# Autodesk Inventor assembly: Case
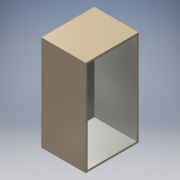
[picture p0: Inventor's stored thumbnail of the model, 180x180]
Saved by Autodesk Inventor 2017 (Build 210142000, 142)
## iProperties
Created: 2016-12-13
Part Number: Case
Document SubType Name: Assembly
Designer: umr
Author: umr
## Documents named in this file (4)
- D:\SeniorProject\Models2\Case\Case.iam
- D:\SeniorProject\Models2\Case\NarrowWall.iam
- D:\SeniorProject\Models2\Case\WideWall.iam
- D:\SeniorProject\Models2\Case\Ceiling.iam
## Components (5 placed, 3 different names)
1. NarrowWall:1 [sub-assembly] — Mate:2, Flush:7, Flush:14, Flush:16, Mate:6, Flush:17, Animation1
2. NarrowWall:2 [sub-assembly] — Flush:12, Flush:13, Animation2
3. WideWall:1 [sub-assembly] — Mate:2, Flush:7, Flush:12, Flush:13, Flush:14, Flush:18, Animation3
4. WideWall:2 [sub-assembly] — Flush:16, Mate:6, Animation1, Animation2
5. Ceiling:1 [sub-assembly] — Flush:17, Flush:18, Animation3
## Relationships (12: Flush 8, Mate 4)
- Mate:2: NarrowWall:1 ↔ WideWall:1
- Flush:7: NarrowWall:1 ↔ WideWall:1
- Flush:12: NarrowWall:2 ↔ WideWall:1
- Flush:13: NarrowWall:2 ↔ WideWall:1
- Flush:14: NarrowWall:1 ↔ WideWall:1
- Flush:16: NarrowWall:1 ↔ WideWall:2
- Mate:6: NarrowWall:1 ↔ WideWall:2
- Flush:17: NarrowWall:1 ↔ Ceiling:1
- Flush:18: WideWall:1 ↔ Ceiling:1
- Animation1 [Flush]: NarrowWall:1 ↔ WideWall:2
- Animation2 [Mate]: NarrowWall:2 ↔ WideWall:2
- Animation3 [Mate]: WideWall:1 ↔ Ceiling:1
